# Autodesk Inventor assembly: Palm_Assembly
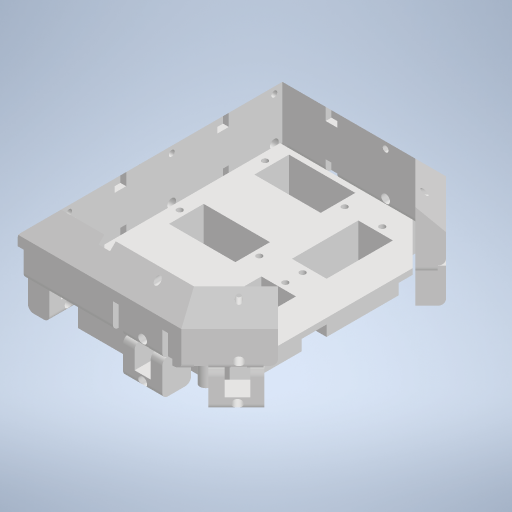
[picture p0: Inventor's stored thumbnail of the model, 512x512]
Saved by Autodesk Inventor 2023 (Build 270158000, 158)
## iProperties
Created: 2023-04-30
Part Number: Palm_Assembly
Document SubType Name: Assembly
Designer: adity
Author: adity
## Documents named in this file (3)
- C:\Users\adity\Downloads\Inventor\Robotic Hand\Palm_Assembly.iam
- C:\Users\adity\Downloads\Inventor\Robotic Hand\Palm_ServoAttachment.ipt
- C:\Users\adity\Downloads\Inventor\Robotic Hand\Palm_FingerAttachment.ipt
## Components (2 placed, 2 different names)
1. Palm_FingerAttachment:1 — Mate:1, Mate:2
2. Palm_ServoAttachment:3 — Mate:1, Mate:2
## Relationships (2: Mate 2)
- Mate:1: Palm_FingerAttachment:1 ↔ Palm_ServoAttachment:3
- Mate:2: Palm_FingerAttachment:1 ↔ Palm_ServoAttachment:3
